# Autodesk Inventor assembly: Valve Assembly
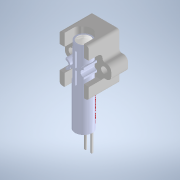
[picture p0: Inventor's stored thumbnail of the model, 180x180]
Saved by Autodesk Inventor 2021 (Build 250183000, 183)
## iProperties
Created: 2020-07-16
Part Number: Valve Assembly
Document SubType Name: Assembly
Designer: jgray
Author: jgray
## Documents named in this file (3)
- M:\Printed Electronics\Gas Sensors\Prototypes\Prototype II -Cartridge Reader V3\Valve Assembly.iam
- M:\Printed Electronics\Gas Sensors\Prototypes\Prototype II -Cartridge Reader V3\clamp1wide.ipt
- M:\Printed Electronics\Gas Sensors\Prototypes\Prototype II -Cartridge Reader V3\LHDA3D00006AA - PRTD - 3Way,2Way - V1.ipt
## Components (2 placed, 2 different names)
1. clamp1wide:1 — Mate:1, Mate:2
2. LHDA3D00006AA - PRTD - 3Way,2Way - V1:1 — Mate:1, Mate:2
## Relationships (2: Mate 2)
- Mate:1: clamp1wide:1 ↔ LHDA3D00006AA - PRTD - 3Way,2Way - V1:1
- Mate:2: clamp1wide:1 ↔ LHDA3D00006AA - PRTD - 3Way,2Way - V1:1
